# Autodesk Inventor assembly: アーム用初段
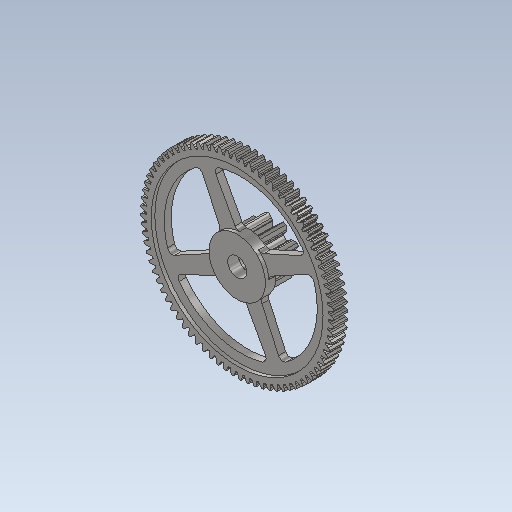
[picture p0: Inventor's stored thumbnail of the model, 512x512]
Saved by Autodesk Inventor 2020.2 (Build 242310000, 310)
## iProperties
Created: 2020-03-15
Part Number: アーム用初段
Document SubType Name: Assembly
Designer: aoyam
Mass: 12.9963 g
Surface Area: 31.0724 cm^2
Volume: 1.65558 cm^3
Density: 7.85 g/cm^3
Author: aoyam
## Documents named in this file (3)
- C:\Users\aoyam\Desktop\SRDC_local\Inventor\二年機\Geminiβ\腕\アーム用初段.iam
- C:\Users\aoyam\Desktop\SRDC_local\Inventor\二年機\Geminiβ\汎用部品\m1歯数9ギアd5.98t5.ipt
- C:\Users\aoyam\Desktop\SRDC_local\Inventor\二年機\Geminiβ\汎用部品\ｍ0.5歯数80焼結ギアd4.ipt
## Components (2 placed, 2 different names)
1. m1歯数9ギアd5.98t5:1 — 挿入:1
2. ｍ0.5歯数80焼結ギアd4:1 — 挿入:1
## Relationships (1: Insert 1)
- 挿入:1 [Insert]: m1歯数9ギアd5.98t5:1 ↔ ｍ0.5歯数80焼結ギアd4:1
